# Autodesk Inventor assembly: _MK-1_Assembly
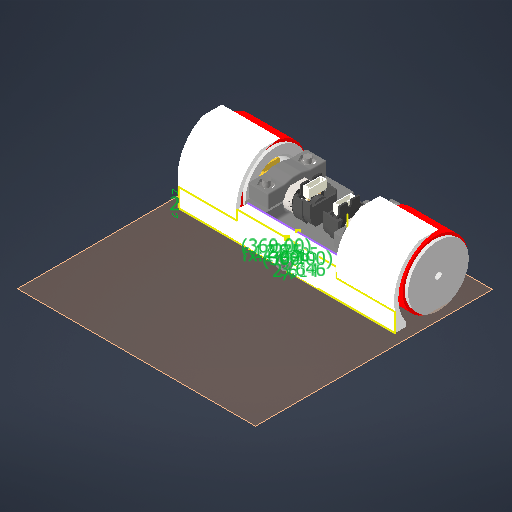
[picture p0: Inventor's stored thumbnail of the model, 512x512]
Saved by Autodesk Inventor 2026.2 (Build 302298010, 298A)
## iProperties
Created: 2026-03-30
Part Number: _MK-1_Assembly
Document SubType Name: Assembly
Designer: zak
Author: zak
## Documents named in this file (14)
- C:\Users\Martin\Pracovní\data\Projekty\Minisumo\Github\NeoSumec-MiniSumo-MECH\_MK-1_\_MK-1_Assembly.iam
- C:\Users\Martin\Pracovní\data\Projekty\Minisumo\Github\NeoSumec-MiniSumo-MECH\_MK-1_\Models\3D_Print\MotorMountBottom.ipt
- C:\Users\Martin\Pracovní\data\Projekty\Minisumo\Github\NeoSumec-MiniSumo-MECH\_MK-1_\Models\3rd-party_comp\Pololu Micro Metal Gearmotor 3D (STEP) Models\With Encoder, Side Connector\mmgm-cb-enc-side-con\mmgm-cb-enc-side-con\mmgm-cb-enc-side-con.ipt
- C:\Users\Martin\Pracovní\data\Projekty\Minisumo\Github\NeoSumec-MiniSumo-MECH\_MK-1_\Models\3D_Print\MotorClamp.ipt
- C:\Users\Martin\Pracovní\data\Projekty\Minisumo\Github\NeoSumec-MiniSumo-MECH\_MK-1_\Models\Metal\Wheel.ipt
- C:\Users\Martin\Pracovní\data\Projekty\Minisumo\Github\NeoSumec-MiniSumo-MECH\_MK-1_\Models\Other technology\silicon bublebum.ipt
- C:\Users\Martin\Pracovní\data\Projekty\Minisumo\Github\NeoSumec-MiniSumo-MECH\_MK-1_\Models\Metal\pipe.ipt
- C:\Users\Martin\Pracovní\data\Projekty\Minisumo\Github\NeoSumec-MiniSumo-MECH\_MK-1_\SpojMat\DIN 934 - M3 x 0,5.ipt
- C:\Users\Martin\Pracovní\data\Projekty\Minisumo\Github\NeoSumec-MiniSumo-MECH\_MK-1_\SpojMat\ISO 14581 - M3x20-4.8.ipt
- C:\Users\Martin\Pracovní\data\Projekty\Minisumo\Github\NeoSumec-MiniSumo-MECH\_MK-1_\SpojMat\ISO 14581 - M3x16-4.8.ipt
- C:\Users\Martin\Pracovní\data\Projekty\Minisumo\Github\NeoSumec-MiniSumo-MECH\_MK-1_\SpojMat\ISO 14580 M3x25-4.8.ipt
- C:\Users\Martin\Pracovní\data\Projekty\Minisumo\Github\NeoSumec-MiniSumo-MECH\_MK-1_\Models\Metal\Knife.ipt
- C:\Users\Martin\Pracovní\data\Projekty\Minisumo\Moje modely k Mk1\main body wheels part.ipt
- C:\Users\Martin\Documents\Inventor\Content Center Files\R2026\en-US\DIN EN ISO 4032\DIN EN ISO 4032 - M3.ipt
## Components (22 placed, 13 different names)
1. MotorMountBottom:1 — Flush:1, Mate:1, Flush:2, Mate:2, Mate:4, Mate:5, Mate:7, Mate:8, Mate:13, Mate:18, Mate:19, Flush:3, Mate:20, Mate:21, Mate:35, Mate:36, Mate:37, Mate:38, Mate:39, Mate:43, Flush:4
2. mmgm-cb-enc-side-con:1 — Flush:2, Mate:2, Mate:3, Mate:9, Mate:10
3. mmgm-cb-enc-side-con:2 — Flush:1, Mate:1, Mate:6, Mate:16, Mate:17
4. MotorClamp:1 — Mate:6, Mate:7, Mate:8, Mate:23, Mate:24, Mate:29, Mate:30, Mate:31
5. MotorClamp:2 — Mate:3, Mate:4, Mate:5, Mate:25, Mate:26, Mate:27, Mate:28, Mate:32, Mate:33
6. Wheel:1 — Mate:14, Mate:15, Mate:16, Mate:17, Mate:18, Flush:5
7. Wheel:2 — Mate:9, Mate:10, Mate:11, Mate:12, Mate:13
8. silicon bublebum:1 — Mate:11, Mate:12
9. silicon bublebum:2 — Mate:14, Mate:15
10. pipe:1 — Mate:19, Flush:3, Mate:40, Mate:41
11. DIN 934 - M3 x 0,5:1 — Mate:29, Mate:30, Mate:31
12. DIN 934 - M3 x 0,5:2 — Mate:28, Mate:32, Mate:33
13. DIN 934 - M3 x 0,5:3 — Mate:25, Mate:26, Mate:27, Mate:34
14. DIN 934 - M3 x 0,5:4 — Mate:22, Mate:23, Mate:24
15. ISO 14581 - M3x20-4.8:1 — Mate:34, Mate:35
16. ISO 14581 - M3x20-4.8:2 — Mate:20, Mate:21, Mate:22
17. ISO 14581 - M3x16-4.8:1 — Mate:36, Mate:37
18. ISO 14581 - M3x16-4.8:2 — Mate:38, Mate:39
19. ISO 14580 M3x25-4.8:1 — Mate:40, Mate:41, Mate:44
20. Knife:2 — Mate:42
21. main body wheels part:1 — Mate:43, Flush:4, Flush:5, Mate:45
22. DIN EN ISO 4032 M3:1 — Mate:44, Mate:45
## Relationships (50: Mate 45, Flush 5)
- Flush:1 (-5 mm): MotorMountBottom:1 ↔ mmgm-cb-enc-side-con:2
- Mate:1: MotorMountBottom:1 ↔ mmgm-cb-enc-side-con:2
- Flush:2 (-5 mm): MotorMountBottom:1 ↔ mmgm-cb-enc-side-con:1
- Mate:2: MotorMountBottom:1 ↔ mmgm-cb-enc-side-con:1
- Mate:3: mmgm-cb-enc-side-con:1 ↔ MotorClamp:2
- Mate:4: MotorMountBottom:1 ↔ MotorClamp:2
- Mate:5: MotorMountBottom:1 ↔ MotorClamp:2
- Mate:6: mmgm-cb-enc-side-con:2 ↔ MotorClamp:1
- Mate:7: MotorMountBottom:1 ↔ MotorClamp:1
- Mate:8: MotorMountBottom:1 ↔ MotorClamp:1
- Mate:9: mmgm-cb-enc-side-con:1 ↔ Wheel:2
- Mate:10 (0.1 mm): mmgm-cb-enc-side-con:1 ↔ Wheel:2
- Mate:11: Wheel:2 ↔ silicon bublebum:1
- Mate:12: Wheel:2 ↔ silicon bublebum:1
- Mate:13 (0.5 mm): MotorMountBottom:1 ↔ Wheel:2
- Mate:14: Wheel:1 ↔ silicon bublebum:2
- Mate:15: Wheel:1 ↔ silicon bublebum:2
- Mate:16: mmgm-cb-enc-side-con:2 ↔ Wheel:1
- Mate:17 (0.25 mm): mmgm-cb-enc-side-con:2 ↔ Wheel:1
- Mate:18 (0.5 mm): MotorMountBottom:1 ↔ Wheel:1
- Mate:19: MotorMountBottom:1 ↔ pipe:1
- Flush:3: MotorMountBottom:1 ↔ pipe:1
- Mate:20: MotorMountBottom:1 ↔ ISO 14581 - M3x20-4.8:2
- Mate:21: MotorMountBottom:1 ↔ ISO 14581 - M3x20-4.8:2
- Mate:22: DIN 934 - M3 x 0,5:4 ↔ ISO 14581 - M3x20-4.8:2
- Mate:23 (0.125 mm): MotorClamp:1 ↔ DIN 934 - M3 x 0,5:4
- Mate:24: MotorClamp:1 ↔ DIN 934 - M3 x 0,5:4
- Mate:25 (0.125 mm): MotorClamp:2 ↔ DIN 934 - M3 x 0,5:3
- Mate:26: MotorClamp:2 ↔ DIN 934 - M3 x 0,5:3
- Mate:27: MotorClamp:2 ↔ DIN 934 - M3 x 0,5:3
- Mate:28: MotorClamp:2 ↔ DIN 934 - M3 x 0,5:2
- Mate:29: MotorClamp:1 ↔ DIN 934 - M3 x 0,5:1
- Mate:30 (0.125 mm): MotorClamp:1 ↔ DIN 934 - M3 x 0,5:1
- Mate:31: MotorClamp:1 ↔ DIN 934 - M3 x 0,5:1
- Mate:32 (0.125 mm): MotorClamp:2 ↔ DIN 934 - M3 x 0,5:2
- Mate:33: MotorClamp:2 ↔ DIN 934 - M3 x 0,5:2
- Mate:34: DIN 934 - M3 x 0,5:3 ↔ ISO 14581 - M3x20-4.8:1
- Mate:35: MotorMountBottom:1 ↔ ISO 14581 - M3x20-4.8:1
- Mate:36: MotorMountBottom:1 ↔ ISO 14581 - M3x16-4.8:1
- Mate:37: MotorMountBottom:1 ↔ ISO 14581 - M3x16-4.8:1
- Mate:38: MotorMountBottom:1 ↔ ISO 14581 - M3x16-4.8:2
- Mate:39: MotorMountBottom:1 ↔ ISO 14581 - M3x16-4.8:2
- Mate:40: pipe:1 ↔ ISO 14580 M3x25-4.8:1
- Mate:41: pipe:1 ↔ ISO 14580 M3x25-4.8:1
- Mate:42: Knife:2
- Mate:43: MotorMountBottom:1 ↔ main body wheels part:1
- Flush:4: MotorMountBottom:1 ↔ main body wheels part:1
- Flush:5: Wheel:1 ↔ main body wheels part:1
- Mate:44: ISO 14580 M3x25-4.8:1 ↔ DIN EN ISO 4032 M3:1
- Mate:45: main body wheels part:1 ↔ DIN EN ISO 4032 M3:1
